# Autodesk Inventor assembly: calosc
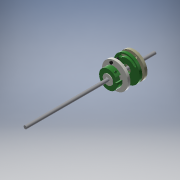
[picture p0: Inventor's stored thumbnail of the model, 180x180]
Saved by Autodesk Inventor 2017 (Build 210142000, 142)
## iProperties
Created: 2021-05-22
Part Number: calosc
Document SubType Name: Assembly
Designer: majch
Author: majch
## Documents named in this file (8)
- E:\inventor\mocowanie\calosc.iam
- E:\inventor\mocowanie\ogolny_walek-013.ipt
- E:\inventor\mocowanie\ogolny_walek.ipt
- E:\inventor\mocowanie\sprzeglo_03.ipt
- E:\inventor\mocowanie\sprzeglo_02.ipt
- E:\inventor\mocowanie\sprzeglo_01.ipt
- E:\inventor\mocowanie\waleczek_do_sprezyn_fi6.ipt
- E:\inventor\mocowanie\sprzeglo_04.ipt
## Components (7 placed, 6 different names)
1. ogolny_walek-013:1 — Mate:1, Mate:2, Mate:3, Mate:8
2. sprzeglo_03:1 — Mate:3, Mate:6, Flush:3, Mate:9
3. sprzeglo_02:1 — Mate:2, Mate:5, Mate:7, Flush:4
4. sprzeglo_01:1 — Mate:1, Mate:7
5. waleczek_do_sprezyn_fi6:1 — Mate:6, Flush:3
6. waleczek_do_sprezyn_fi6:3 — Mate:5, Flush:4
7. sprzeglo_04:1 — Mate:8, Mate:9
## Relationships (10: Mate 8, Flush 2)
- Mate:1: ogolny_walek-013:1 ↔ sprzeglo_01:1
- Mate:2: ogolny_walek-013:1 ↔ sprzeglo_02:1
- Mate:3: ogolny_walek-013:1 ↔ sprzeglo_03:1
- Mate:5: sprzeglo_02:1 ↔ waleczek_do_sprezyn_fi6:3
- Mate:6: sprzeglo_03:1 ↔ waleczek_do_sprezyn_fi6:1
- Flush:3: sprzeglo_03:1 ↔ waleczek_do_sprezyn_fi6:1
- Mate:7: sprzeglo_02:1 ↔ sprzeglo_01:1
- Flush:4: sprzeglo_02:1 ↔ waleczek_do_sprezyn_fi6:3
- Mate:8: ogolny_walek-013:1 ↔ sprzeglo_04:1
- Mate:9: sprzeglo_03:1 ↔ sprzeglo_04:1
